# Autodesk Inventor assembly: robot new
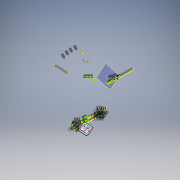
[picture p0: Inventor's stored thumbnail of the model, 180x180]
Saved by Autodesk Inventor 2017 (Build 210142000, 142)
## iProperties
Created: 2017-02-25
Part Number: robot new
Document SubType Name: Assembly
Designer: Jess
Author: Jess
## Documents named in this file (11)
- C:\Users\Jess\Documents\Parts for new robot\robot new.iam
- C:\Users\Jess\Documents\rev extrusion 17 in.ipt
- C:\Users\Jess\Documents\reverend extrusion 9 in.ipt
- C:\Users\Jess\Documents\Axle hub.ipt
- C:\Users\Jess\Documents\Mecanum 4'' left.iam
- C:\Users\Jess\Documents\Parts for new robot\mecanumm 4'' right.iam
- C:\Users\Jess\Documents\Parts for new robot\axle 100mm.ipt
- C:\Users\Jess\Documents\Parts for new robot\32 tooth sprocket tetrix.ipt
- C:\Users\Jess\Documents\Parts for new robot\ftc conversion plate.ipt
- C:\Users\Jess\Documents\Parts for new robot\24 tooth sprocket tetrix.ipt
- C:\Users\Jess\Documents\Parts for new robot\crappy frame that isnt constrained.iam
## Components (33 placed, 10 different names)
1. rev extrusion 17 in:1
2. rev extrusion 17 in:2
3. reverend extrusion 9 in:1
4. Axle hub:1
5. Axle hub:2 — Insert:5, Insert:7
6. Axle hub:3 — Insert:4, Insert:6
7. Axle hub:4
8. Axle hub:5
9. Axle hub:6
10. Axle hub:7 — Insert:2, Insert:9
11. Axle hub:8 — Insert:3, Insert:8
12. Mecanum 4'' left:1 [sub-assembly] — Mate:15, Mate:16, Mate:17
13. Mecanum 4'' left:2 [sub-assembly] — Mate:12, Mate:13, Mate:14
14. mecanumm 4'' right:1 [sub-assembly] — Mate:9, Mate:10, Mate:11
15. mecanumm 4'' right:2 [sub-assembly] — Mate:6, Mate:7, Mate:8
16. axle 100mm:1 — Insert:6, Insert:11
17. axle 100mm:2 — Insert:8, Insert:12
18. axle 100mm:3 — Insert:9, Insert:13
19. axle 100mm:4 — Insert:7, Insert:10
20. 32 tooth sprocket tetrix:1
21. 32 tooth sprocket tetrix:2
22. 32 tooth sprocket tetrix:3
23. 32 tooth sprocket tetrix:4
24. reverend extrusion 9 in:2 — Flush:1
25. ftc conversion plate:1 — Mate:15, Mate:16, Mate:17, Mate:27, Mate:28, Mate:29
26. ftc conversion plate:2 — Mate:9, Mate:10, Mate:11, Mate:24, Mate:25, Mate:26
27. ftc conversion plate:3 — Mate:12, Mate:13, Mate:14, Mate:18, Mate:19, Mate:20
28. ftc conversion plate:4 — Mate:6, Mate:7, Mate:8, Mate:21, Mate:22, Mate:23
29. 24 tooth sprocket tetrix:1 — Mate:27, Mate:28, Mate:29, Insert:3
30. 24 tooth sprocket tetrix:2 — Mate:24, Mate:25, Mate:26, Insert:5
31. 24 tooth sprocket tetrix:3 — Mate:21, Mate:22, Mate:23, Insert:4
32. 24 tooth sprocket tetrix:4 — Mate:18, Mate:19, Mate:20, Insert:2
33. crappy frame that isnt constrained:1 [sub-assembly] — Insert:10, Insert:11, Insert:12, Insert:13
## Relationships (37: Mate 24, Insert 12, Flush 1)
- Flush:1: reverend extrusion 9 in:2
- Mate:6: mecanumm 4'' right:2 ↔ ftc conversion plate:4
- Mate:7: mecanumm 4'' right:2 ↔ ftc conversion plate:4
- Mate:8: mecanumm 4'' right:2 ↔ ftc conversion plate:4
- Mate:9: mecanumm 4'' right:1 ↔ ftc conversion plate:2
- Mate:10: mecanumm 4'' right:1 ↔ ftc conversion plate:2
- Mate:11: mecanumm 4'' right:1 ↔ ftc conversion plate:2
- Mate:12: Mecanum 4'' left:2 ↔ ftc conversion plate:3
- Mate:13: Mecanum 4'' left:2 ↔ ftc conversion plate:3
- Mate:14: Mecanum 4'' left:2 ↔ ftc conversion plate:3
- Mate:15: Mecanum 4'' left:1 ↔ ftc conversion plate:1
- Mate:16: Mecanum 4'' left:1 ↔ ftc conversion plate:1
- Mate:17: Mecanum 4'' left:1 ↔ ftc conversion plate:1
- Mate:18: ftc conversion plate:3 ↔ 24 tooth sprocket tetrix:4
- Mate:19: ftc conversion plate:3 ↔ 24 tooth sprocket tetrix:4
- Mate:20: ftc conversion plate:3 ↔ 24 tooth sprocket tetrix:4
- Mate:21: ftc conversion plate:4 ↔ 24 tooth sprocket tetrix:3
- Mate:22: ftc conversion plate:4 ↔ 24 tooth sprocket tetrix:3
- Mate:23: ftc conversion plate:4 ↔ 24 tooth sprocket tetrix:3
- Mate:24: ftc conversion plate:2 ↔ 24 tooth sprocket tetrix:2
- Mate:25: ftc conversion plate:2 ↔ 24 tooth sprocket tetrix:2
- Mate:26: ftc conversion plate:2 ↔ 24 tooth sprocket tetrix:2
- Mate:27: ftc conversion plate:1 ↔ 24 tooth sprocket tetrix:1
- Mate:28: ftc conversion plate:1 ↔ 24 tooth sprocket tetrix:1
- Mate:29: ftc conversion plate:1 ↔ 24 tooth sprocket tetrix:1
- Insert:2: Axle hub:7 ↔ 24 tooth sprocket tetrix:4
- Insert:3: Axle hub:8 ↔ 24 tooth sprocket tetrix:1
- Insert:4: Axle hub:3 ↔ 24 tooth sprocket tetrix:3
- Insert:5: Axle hub:2 ↔ 24 tooth sprocket tetrix:2
- Insert:6 (-34.29 mm): Axle hub:3 ↔ axle 100mm:1
- Insert:7 (-25.4 mm): Axle hub:2 ↔ axle 100mm:4
- Insert:8 (-66.04 mm): Axle hub:8 ↔ axle 100mm:2
- Insert:9 (-25.4 mm): Axle hub:7 ↔ axle 100mm:3
- Insert:10 (-66.04 mm): axle 100mm:4 ↔ crappy frame that isnt constrained:1
- Insert:11 (-57.15 mm): axle 100mm:1 ↔ crappy frame that isnt constrained:1
- Insert:12 (-25.4 mm): axle 100mm:2 ↔ crappy frame that isnt constrained:1
- Insert:13 (-66.04 mm): axle 100mm:3 ↔ crappy frame that isnt constrained:1
